# Autodesk Inventor assembly: Assembly_cajativa
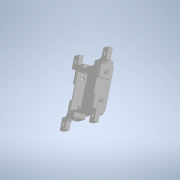
[picture p0: Inventor's stored thumbnail of the model, 180x180]
Saved by Autodesk Inventor 2022 (Build 260153000, 153)
## iProperties
Created: 2022-03-18
Part Number: Assembly_cajativa
Document SubType Name: Assembly
Designer: jrdia
Author: jrdia
## Documents named in this file (5)
- D:\Semestre_9\Diseño_Innovación_1\mini1_diseno\archivos_stl\Assembly_cajativa.iam
- D:\Semestre_9\Diseño_Innovación_1\mini1_diseno\pared1_cajativa.ipt
- D:\Semestre_9\Diseño_Innovación_1\mini1_diseno\pared2_cajativa.ipt
- D:\Semestre_9\Diseño_Innovación_1\mini1_diseno\tapa_tiva.ipt
- D:\Semestre_9\Diseño_Innovación_1\mini1_diseno\escuadra_caja.ipt
## Components (9 placed, 4 different names)
1. pared1_cajativa:1 — Mate:7, Mate:8, Mate:9, Mate:11, Mate:14, Mate:22, Mate:23
2. pared1_cajativa:2 — Mate:1, Mate:2, Mate:3, Mate:4, Mate:5, Mate:6, Mate:10, Mate:16, Mate:20
3. pared2_cajativa:1 — Mate:4, Mate:5, Mate:6, Mate:7, Mate:13, Mate:15, Mate:17, Mate:18
4. pared2_cajativa:2 — Mate:1, Mate:2, Mate:3, Mate:8, Mate:9, Mate:12, Mate:19, Mate:21, Mate:24
5. tapa_tiva:1 — Mate:10, Mate:11, Mate:12
6. escuadra_caja:1 — Mate:13, Mate:14, Mate:15
7. escuadra_caja:2 — Mate:16, Mate:17, Mate:18
8. escuadra_caja:3 — Mate:19, Mate:20, Mate:21
9. escuadra_caja:4 — Mate:22, Mate:23, Mate:24
## Relationships (24: Mate 24)
- Mate:1: pared1_cajativa:2 ↔ pared2_cajativa:2
- Mate:2: pared1_cajativa:2 ↔ pared2_cajativa:2
- Mate:3: pared1_cajativa:2 ↔ pared2_cajativa:2
- Mate:4: pared1_cajativa:2 ↔ pared2_cajativa:1
- Mate:5: pared1_cajativa:2 ↔ pared2_cajativa:1
- Mate:6: pared1_cajativa:2 ↔ pared2_cajativa:1
- Mate:7: pared1_cajativa:1 ↔ pared2_cajativa:1
- Mate:8: pared1_cajativa:1 ↔ pared2_cajativa:2
- Mate:9: pared1_cajativa:1 ↔ pared2_cajativa:2
- Mate:10: pared1_cajativa:2 ↔ tapa_tiva:1
- Mate:11: pared1_cajativa:1 ↔ tapa_tiva:1
- Mate:12: pared2_cajativa:2 ↔ tapa_tiva:1
- Mate:13: pared2_cajativa:1 ↔ escuadra_caja:1
- Mate:14: pared1_cajativa:1 ↔ escuadra_caja:1
- Mate:15: pared2_cajativa:1 ↔ escuadra_caja:1
- Mate:16: pared1_cajativa:2 ↔ escuadra_caja:2
- Mate:17: pared2_cajativa:1 ↔ escuadra_caja:2
- Mate:18: pared2_cajativa:1 ↔ escuadra_caja:2
- Mate:19: pared2_cajativa:2 ↔ escuadra_caja:3
- Mate:20: pared1_cajativa:2 ↔ escuadra_caja:3
- Mate:21: pared2_cajativa:2 ↔ escuadra_caja:3
- Mate:22: pared1_cajativa:1 ↔ escuadra_caja:4
- Mate:23: pared1_cajativa:1 ↔ escuadra_caja:4
- Mate:24: pared2_cajativa:2 ↔ escuadra_caja:4
